# Autodesk Inventor assembly: ASY TKS 3510 FDS way7
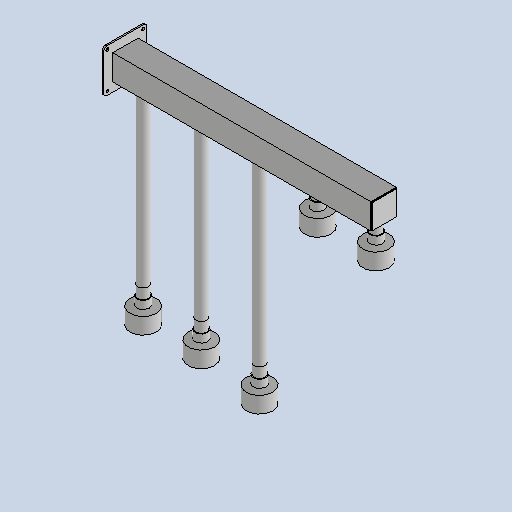
[picture p0: Inventor's stored thumbnail of the model, 512x512]
Saved by Autodesk Inventor 2025 (Build 290162010, 162A)
## iProperties
Created: 2025-07-02
Part Number: ASY TKS 3510 FDS way7
Document SubType Name: Assembly
Designer: user
Author: user
## Documents named in this file (8)
- C:\Users\admin\Yandex.Disk\home pc\Inventor\TKS-Tarko-Sale\BOTTOM DS\ASY TKS 3510 FDS way7.iam
- C:\Users\admin\Yandex.Disk\home pc\Inventor\TKS-Tarko-Sale\BOTTOM DS\TKS 3511 FDS way tube 7.ipt
- C:\Users\admin\Yandex.Disk\home pc\Inventor\TKS-Tarko-Sale\BOTTOM DS\TKS dummy filter element.ipt
- C:\Users\admin\Yandex.Disk\home pc\Inventor\TKS-Tarko-Sale\BOTTOM DS\TKS dummy pipe nippel.ipt
- C:\Users\admin\Yandex.Disk\home pc\Inventor\TKS-Tarko-Sale\BOTTOM DS\TKS 3542 FDS thread  tube2.ipt
- C:\Users\admin\Yandex.Disk\home pc\Inventor\TKS-Tarko-Sale\BOTTOM DS\TKS 3541 FDS thread  tube1.ipt
- C:\Users\admin\Yandex.Disk\home pc\Inventor\TKS-Tarko-Sale\BOTTOM DS\TKS 3531 FDS Way FLANGE.ipt
- C:\Users\admin\Yandex.Disk\home pc\Inventor\TKS-Tarko-Sale\BOTTOM DS\TKS 3532 FDS way cup.ipt
## Components (16 placed, 7 different names)
1. TKS 3511 FDS way tube 7.ipt:1 — Rigid:13, Rigid:15, Rotational:2
2. TKS dummy filter element.ipt:1
3. TKS dummy pipe nippel.ipt:1
4. TKS dummy filter element.ipt:2
5. TKS dummy pipe nippel.ipt:2 — Rotational:1
6. TKS 3542 FDS thread  tube2.ipt:1
7. TKS dummy filter element.ipt:3
8. TKS dummy pipe nippel.ipt:3
9. TKS 3541 FDS thread  tube1.ipt:1
10. TKS dummy filter element.ipt:4
11. TKS dummy pipe nippel.ipt:4
12. TKS 3531 FDS Way FLANGE.ipt:1
13. TKS 3532 FDS way cup.ipt:1 — Rigid:13
14. TKS dummy filter element.ipt:5
15. TKS dummy pipe nippel.ipt:5 — Rigid:15
16. TKS 3542 FDS thread  tube2.ipt:2 — Rotational:1, Rotational:2
## Relationships (15: WeldJoint 13, RevoluteJoint 2)
- [WeldJoint]: TKS dummy filter element.ipt:1 ↔ TKS dummy pipe nippel.ipt:1
- [WeldJoint]: TKS 3511 FDS way tube 7.ipt:1 ↔ TKS dummy pipe nippel.ipt:1
- [WeldJoint]: TKS dummy filter element.ipt:2 ↔ TKS dummy pipe nippel.ipt:2
- [WeldJoint]: TKS dummy filter element.ipt:3 ↔ TKS dummy pipe nippel.ipt:3
- [WeldJoint]: TKS 3542 FDS thread  tube2.ipt:1 ↔ TKS dummy pipe nippel.ipt:3
- [WeldJoint]: TKS dummy filter element.ipt:4 ↔ TKS dummy pipe nippel.ipt:4
- [WeldJoint]: TKS 3541 FDS thread  tube1.ipt:1 ↔ TKS dummy pipe nippel.ipt:4
- [WeldJoint]: TKS 3511 FDS way tube 7.ipt:1 ↔ TKS 3542 FDS thread  tube2.ipt:1
- [WeldJoint]: TKS 3511 FDS way tube 7.ipt:1 ↔ TKS 3541 FDS thread  tube1.ipt:1
- [WeldJoint] (-2 mm): TKS 3511 FDS way tube 7.ipt:1 ↔ TKS 3531 FDS Way FLANGE.ipt:1
- Rigid:13 [WeldJoint]: TKS 3511 FDS way tube 7.ipt:1 ↔ TKS 3532 FDS way cup.ipt:1
- [WeldJoint]: TKS dummy filter element.ipt:5 ↔ TKS dummy pipe nippel.ipt:5
- Rigid:15 [WeldJoint]: TKS 3511 FDS way tube 7.ipt:1 ↔ TKS dummy pipe nippel.ipt:5
- Rotational:1 [RevoluteJoint]: TKS dummy pipe nippel.ipt:2 ↔ TKS 3542 FDS thread  tube2.ipt:2
- Rotational:2 [RevoluteJoint]: TKS 3511 FDS way tube 7.ipt:1 ↔ TKS 3542 FDS thread  tube2.ipt:2
## Named parameters: d33_d31 = 0 mm, d37_d34_d31 = 0 mm, d43_d40_d37_d34_d31 = 0 mm, d44_d41 = 0 mm, d47_d45_d43_d40_d37_d34_d31 = 0 mm, d48_d46 = 0 mm, d13_d47_d45_d43_d40_d37_d34_d31 = 0 mm
